# Autodesk Inventor assembly: Ensamble
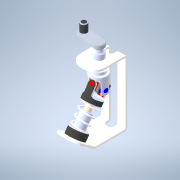
[picture p0: Inventor's stored thumbnail of the model, 180x180]
Saved by Autodesk Inventor 2021 (Build 250183000, 183)
## iProperties
Created: 2021-03-19
Part Number: Ensamble
Document SubType Name: Assembly
Designer: trejo
Author: trejo
## Documents named in this file (10)
- C:\Users\trejo\Documents\Octavo Cuatrimestre\3D Design\homework\Actividad 5\Manivela\Ensamble.iam
- C:\Users\trejo\Documents\Octavo Cuatrimestre\3D Design\homework\Actividad 5\Manivela\SHEET METAL BRACKET.ipt
- C:\Users\trejo\Documents\Octavo Cuatrimestre\3D Design\homework\Actividad 5\Manivela\YOKE_MALE.ipt
- C:\Users\trejo\Documents\Octavo Cuatrimestre\3D Design\homework\Actividad 5\Manivela\HANDLE.ipt
- C:\Users\trejo\Documents\Octavo Cuatrimestre\3D Design\homework\Actividad 5\Manivela\HANDLE_TOP.ipt
- C:\Users\trejo\Documents\Octavo Cuatrimestre\3D Design\homework\Actividad 5\Manivela\SPIDER HINGE.ipt
- C:\Users\trejo\Documents\Octavo Cuatrimestre\3D Design\homework\Actividad 5\Manivela\BLUE_PIN.ipt
- C:\Users\trejo\Documents\Octavo Cuatrimestre\3D Design\homework\Actividad 5\Manivela\YOKE_FEMALE.ipt
- C:\Users\trejo\Documents\Octavo Cuatrimestre\3D Design\homework\Actividad 5\Manivela\RED_PIN.ipt
- C:\Users\trejo\Documents\Octavo Cuatrimestre\3D Design\homework\Actividad 5\Manivela\FASTNER.ipt
## Components (11 placed, 9 different names)
1. SHEET METAL BRACKET:1 — Mate:1, Mate:6
2. YOKE_MALE:1 — Mate:1, Mate:3, Mate:4, Mate:5, Rotational:1, Rigid:2, Rigid:3
3. HANDLE:1 — Mate:3, Mate:4, Mate:5, Rigid:1
4. HANDLE_TOP:1 — Rigid:1
5. SPIDER HINGE:1 — Rotational:1, Rotational:2, Rotational:3, Rotational:4
6. BLUE_PIN:1 — Rigid:2
7. BLUE_PIN:2 — Rigid:3
8. YOKE_FEMALE:1 — Rotational:2, Rigid:4, Mate:6
9. RED_PIN:1 — Rigid:4
10. FASTNER:1 — Rotational:3
11. FASTNER:2 — Rotational:4
## Relationships (13: Mate 5, WeldJoint 4, RevoluteJoint 4)
- Mate:1: SHEET METAL BRACKET:1 ↔ YOKE_MALE:1
- Mate:3: YOKE_MALE:1 ↔ HANDLE:1
- Mate:4: YOKE_MALE:1 ↔ HANDLE:1
- Mate:5: YOKE_MALE:1 ↔ HANDLE:1
- Rigid:1 [WeldJoint]: HANDLE:1 ↔ HANDLE_TOP:1
- Rotational:1 [RevoluteJoint]: YOKE_MALE:1 ↔ SPIDER HINGE:1
- Rigid:2 [WeldJoint]: YOKE_MALE:1 ↔ BLUE_PIN:1
- Rigid:3 [WeldJoint]: YOKE_MALE:1 ↔ BLUE_PIN:2
- Rotational:2 [RevoluteJoint]: SPIDER HINGE:1 ↔ YOKE_FEMALE:1
- Rigid:4 [WeldJoint]: YOKE_FEMALE:1 ↔ RED_PIN:1
- Mate:6: SHEET METAL BRACKET:1 ↔ YOKE_FEMALE:1
- Rotational:3 [RevoluteJoint]: SPIDER HINGE:1 ↔ FASTNER:1
- Rotational:4 [RevoluteJoint]: SPIDER HINGE:1 ↔ FASTNER:2
